# Autodesk Inventor assembly: Battery Cart Storage Assembly
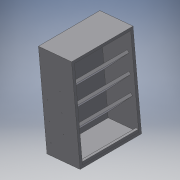
[picture p0: Inventor's stored thumbnail of the model, 180x180]
Saved by Autodesk Inventor 2018 (Build 220112000, 112)
## iProperties
Created: 2018-12-10
Part Number: Battery Cart Storage Assembly
Document SubType Name: Assembly
Designer: Gabriel
Author: Gabriel
## Documents named in this file (4)
- C:\Users\Gabriel\Documents\GitHub\2019CAD\Gab Battery Cart\Battery Cart Storage Assembly.iam
- C:\Users\Gabriel\Documents\GitHub\2019CAD\Gab Battery Cart\Cart Box.ipt
- C:\Users\Gabriel\Documents\GitHub\2019CAD\Gab Battery Cart\Cart Shelf.ipt
- C:\Users\Gabriel\Documents\GitHub\2019CAD\Gab Battery Cart\Bottom Bumper.ipt
## Components (5 placed, 3 different names)
1. Cart Box:1 — Mate:1, Mate:2, Mate:3, Mate:4, Mate:5, Mate:6, Mate:7
2. Cart Shelf:2 — Mate:4, Mate:5
3. Cart Shelf:3 — Mate:2, Mate:3
4. Bottom Bumper:1 — Mate:6, Mate:7
5. Cart Shelf:4 — Mate:1
## Relationships (7: Mate 7)
- Mate:1: Cart Box:1 ↔ Cart Shelf:4
- Mate:2: Cart Box:1 ↔ Cart Shelf:3
- Mate:3: Cart Box:1 ↔ Cart Shelf:3
- Mate:4: Cart Box:1 ↔ Cart Shelf:2
- Mate:5: Cart Box:1 ↔ Cart Shelf:2
- Mate:6: Cart Box:1 ↔ Bottom Bumper:1
- Mate:7: Cart Box:1 ↔ Bottom Bumper:1
